# Autodesk Inventor assembly: Arm 2.0 Assembly
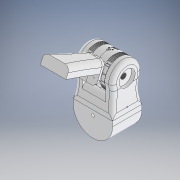
[picture p0: Inventor's stored thumbnail of the model, 180x180]
Saved by Autodesk Inventor 2017 SP1 (Build 210196100, 196)
## iProperties
Created: 2017-09-28
Part Number: Arm 2.0 Assembly
Document SubType Name: Assembly
Designer: Zach
Author: Zach
## Documents named in this file (12)
- C:\Users\Zach\Documents\GitHub\tr1\src\Body\Arm 2.0 Assembly\Arm 2.0 Assembly.iam
- C:\Users\Zach\Documents\GitHub\tr1\src\Body\Arm 2.0 Assembly\AA001.ipt
- C:\Users\Zach\Documents\GitHub\tr1\src\Body\Arm 2.0 Assembly\Steel Rod 8mm x 135mm.ipt
- C:\Users\Zach\Documents\GitHub\tr1\lib\22x8x8mm Bearing.ipt
- C:\Users\Zach\Documents\GitHub\tr1\src\Body\Arm 2.0 Assembly\AA002.ipt
- C:\Users\Zach\Documents\GitHub\tr1\src\Body\Arm 2.0 Assembly\AA003.ipt
- C:\Users\Zach\Documents\GitHub\tr1\src\Body\Arm 2.0 Assembly\AA004.ipt
- C:\Users\Zach\Documents\GitHub\tr1\src\Body\Arm 2.0 Assembly\AA005.ipt
- C:\Users\Zach\Documents\GitHub\tr1\src\Body\Arm 2.0 Assembly\AA006.ipt
- C:\Users\Zach\Documents\GitHub\tr1\src\Body\Arm 2.0 Assembly\AA007.ipt
- C:\Users\Zach\Documents\GitHub\tr1\lib\QS12MM250\QS12MM250.ipt
- C:\Users\Zach\Documents\GitHub\tr1\src\Body\Arm 2.0 Assembly\AA008.ipt
## Components (13 placed, 11 different names)
1. AA001:1 — Mate:1, Mate:3, Flush:1, Mate:4, Flush:2, Mate:7, Mate:9, Mate:10, Mate:11
2. Steel Rod 8mm x 135mm:1 — Mate:1, Flush:3, Mate:6
3. 22x8x8mm Bearing:1 — Mate:3, Flush:1, Flush:3
4. 22x8x8mm Bearing:2 — Mate:4, Flush:2
5. AA002:2 — Flush:4, Mate:5, Mate:8, Mate:14, Mate:28, Mate:29
6. AA003:1 — Flush:4, Mate:5, Mate:6, Mate:7, Mate:8, Mate:27
7. AA004:1 — Mate:9, Mate:10, Mate:11, Mate:12, Mate:13, Mate:15, Mate:23, Mate:26
8. AA005:1 — Mate:16, Mate:17, Mate:18, Mate:26
9. AA006:1 — Mate:21, Mate:22, Mate:24, Mate:25
10. AA007:1 — Mate:16, Mate:17, Mate:18, Mate:19, Mate:20
11. AA007:2 — Mate:19, Mate:20, Mate:21, Mate:22
12. QS12MM250:1 — Mate:23, Mate:24, Mate:25
13. AA008:1 — Mate:27, Mate:28, Mate:29
## Relationships (32: Mate 28, Flush 4)
- Mate:1: AA001:1 ↔ Steel Rod 8mm x 135mm:1
- Mate:3: AA001:1 ↔ 22x8x8mm Bearing:1
- Flush:1: AA001:1 ↔ 22x8x8mm Bearing:1
- Mate:4: AA001:1 ↔ 22x8x8mm Bearing:2
- Flush:2: AA001:1 ↔ 22x8x8mm Bearing:2
- Flush:3 (-2.5 mm): Steel Rod 8mm x 135mm:1 ↔ 22x8x8mm Bearing:1
- Flush:4: AA002:2 ↔ AA003:1
- Mate:5: AA002:2 ↔ AA003:1
- Mate:6: Steel Rod 8mm x 135mm:1 ↔ AA003:1
- Mate:7 (0.75 mm): AA001:1 ↔ AA003:1
- Mate:8: AA002:2 ↔ AA003:1
- Mate:9: AA001:1 ↔ AA004:1
- Mate:10: AA001:1 ↔ AA004:1
- Mate:11: AA001:1 ↔ AA004:1
- Mate:12: AA004:1
- Mate:13: AA004:1
- Mate:14: AA002:2
- Mate:15: AA004:1
- Mate:16: AA005:1 ↔ AA007:1
- Mate:17: AA005:1 ↔ AA007:1
- Mate:18: AA005:1 ↔ AA007:1
- Mate:19: AA007:1 ↔ AA007:2
- Mate:20: AA007:1 ↔ AA007:2
- Mate:21: AA006:1 ↔ AA007:2
- Mate:22: AA006:1 ↔ AA007:2
- Mate:23: AA004:1 ↔ QS12MM250:1
- Mate:24: AA006:1 ↔ QS12MM250:1
- Mate:25: AA006:1 ↔ QS12MM250:1
- Mate:26: AA004:1 ↔ AA005:1
- Mate:27: AA003:1 ↔ AA008:1
- Mate:28: AA002:2 ↔ AA008:1
- Mate:29: AA002:2 ↔ AA008:1
